# Autodesk Inventor assembly: Ball Shifter Shaft assy short output
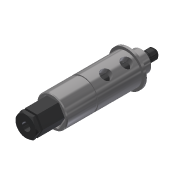
[picture p0: Inventor's stored thumbnail of the model, 180x180]
Saved by Autodesk Inventor 2013 (Build 170138000, 138)
## iProperties
Created: 2013-04-08
Part Number: Ball Shifter Shaft assy short output
Document SubType Name: Assembly
Designer: Niemitalo_Dan
Author: Niemitalo_Dan
## Documents named in this file (4)
- H:\Nemo\Documents\Robotics\COTS Parts\Ballshifter\Ball Shifter Shaft assy short output.iam
- H:\Nemo\Documents\Robotics\COTS Parts\Ballshifter\BallShifter ball housing.ipt
- H:\Nemo\Documents\Robotics\COTS Parts\Ballshifter\Ball shifting shaft.ipt
- H:\Nemo\Documents\Robotics\COTS Parts\Ballshifter\Ballshifter Short Output Shaft.ipt
## Components (3 placed, 3 different names)
1. BallShifter ball housing:1 — Mate:1, Flush:1, Mate:2, Mate:3, Angle:1
2. Ball shifting shaft:1 — Mate:1, Flush:1
3. Ballshifter Short Output Shaft:1 — Mate:2, Mate:3, Angle:1
## Relationships (5: Mate 3, Flush 1, Angle 1)
- Mate:1: BallShifter ball housing:1 ↔ Ball shifting shaft:1
- Flush:1 (8.382 mm): BallShifter ball housing:1 ↔ Ball shifting shaft:1
- Mate:2: BallShifter ball housing:1 ↔ Ballshifter Short Output Shaft:1
- Mate:3: BallShifter ball housing:1 ↔ Ballshifter Short Output Shaft:1
- Angle:1 (0 deg): BallShifter ball housing:1 ↔ Ballshifter Short Output Shaft:1
